# Autodesk Inventor assembly: リンク_6_1
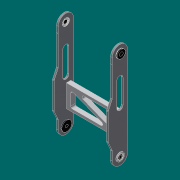
[picture p0: Inventor's stored thumbnail of the model, 180x180]
Saved by Autodesk Inventor 2016 (Build 200138000, 138)
## iProperties
Created: 2016-08-23
Part Number: リンク_6_1
Material: 一般
Document SubType Name: Assembly
Designer: hiro
Mass: 25.4181 g
Surface Area: 148.711 cm^2
Volume: 11.4997 cm^3
Density: 2.21034 g/cm^3
Author: hiro
## Documents named in this file (6)
- C:\Users\hiro\Documents\kenkyuu\二足\二足ver6.0\下半身_160823\リンク\リンク_6_1.iam
- C:\Users\hiro\Documents\kenkyuu\二足\二足ver6.0\既製品\NSK_RB_MF85ZZ\MF85ZZ.iam
- C:\Users\hiro\Documents\kenkyuu\二足\二足ver6.0\下半身\リンク\スペーサ\足首_スペーサ_1_1.ipt
- C:\Users\hiro\Documents\kenkyuu\二足\二足ver6.0\既製品\新規購入\D4050-9120B.ipt
- C:\Users\hiro\Documents\kenkyuu\二足\二足ver6.0\下半身_160823\リンク\リンク_メインフレーム_6_3.ipt
- C:\Users\hiro\Documents\kenkyuu\二足\二足ver6.0\下半身_160823\リンク\リンク_サブフレーム_6_1.ipt
## Components (11 placed, 5 different names)
1. MF85ZZ:1 [sub-assembly] — 挿入:28
2. MF85ZZ:2 [sub-assembly] — 挿入:27
3. 足首_スペーサ_1_1:1
4. 足首_スペーサ_1_1:2
5. MF85ZZ:3 [sub-assembly] — 挿入:19, 挿入:29
6. MF85ZZ:4 [sub-assembly] — 挿入:18, 挿入:26
7. D4050-9120B:1 — 挿入:18
8. D4050-9120B:2 — 挿入:19
9. リンク_メインフレーム_6_3:1 — 挿入:28, 挿入:29, 挿入:30, 挿入:31, 挿入:32
10. リンク_メインフレーム_6_3:2 — 挿入:26, 挿入:27, 挿入:33, 挿入:34, 挿入:35
11. リンク_サブフレーム_6_1:1 — 挿入:30, 挿入:31, 挿入:32, 挿入:33, 挿入:34, 挿入:35
## Relationships (12: Insert 12)
- 挿入:18 [Insert]: MF85ZZ:4 ↔ D4050-9120B:1
- 挿入:19 [Insert]: MF85ZZ:3 ↔ D4050-9120B:2
- 挿入:26 [Insert]: MF85ZZ:4 ↔ リンク_メインフレーム_6_3:2
- 挿入:27 [Insert]: MF85ZZ:2 ↔ リンク_メインフレーム_6_3:2
- 挿入:28 [Insert]: MF85ZZ:1 ↔ リンク_メインフレーム_6_3:1
- 挿入:29 [Insert]: MF85ZZ:3 ↔ リンク_メインフレーム_6_3:1
- 挿入:30 [Insert]: リンク_メインフレーム_6_3:1 ↔ リンク_サブフレーム_6_1:1
- 挿入:31 [Insert]: リンク_メインフレーム_6_3:1 ↔ リンク_サブフレーム_6_1:1
- 挿入:32 [Insert]: リンク_メインフレーム_6_3:1 ↔ リンク_サブフレーム_6_1:1
- 挿入:33 [Insert]: リンク_メインフレーム_6_3:2 ↔ リンク_サブフレーム_6_1:1
- 挿入:34 [Insert]: リンク_メインフレーム_6_3:2 ↔ リンク_サブフレーム_6_1:1
- 挿入:35 [Insert]: リンク_メインフレーム_6_3:2 ↔ リンク_サブフレーム_6_1:1
